# Autodesk Inventor assembly: pat
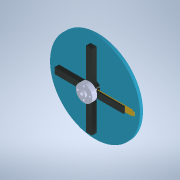
[picture p0: Inventor's stored thumbnail of the model, 180x180]
Saved by Autodesk Inventor 2022 (Build 260153000, 153)
## iProperties
Created: 2022-02-27
Part Number: pat
Document SubType Name: Assembly
Designer: Oana
Author: Oana
## Documents named in this file (4)
- D:\salvari\aplicatii-proiecte\infoeducatia 2022\proiectare\pat_scanare\pat.iam
- D:\salvari\aplicatii-proiecte\infoeducatia 2022\proiectare\pat_scanare\pat.ipt
- D:\salvari\aplicatii-proiecte\infoeducatia 2022\proiectare\pat_scanare\suport + senzor.iam
- D:\salvari\aplicatii-proiecte\infoeducatia 2022\proiectare\piese\39172_txm-axle hub with set screw (1).ipt
## Components (3 placed, 3 different names)
1. pat:1 — Rotational:1
2. suport + senzor:1 [sub-assembly] — Rotational:1, Rotational:2
3. 39172_txm-axle hub with set screw (1):1 — Rotational:2
## Relationships (2: RevoluteJoint 2)
- Rotational:1 [RevoluteJoint]: pat:1 ↔ suport + senzor:1
- Rotational:2 [RevoluteJoint]: suport + senzor:1 ↔ 39172_txm-axle hub with set screw (1):1
